# Autodesk Inventor assembly: leg_motor_moudle_MIR
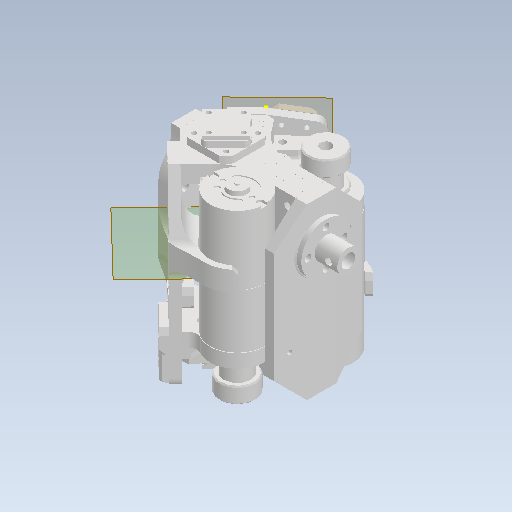
[picture p0: Inventor's stored thumbnail of the model, 512x512]
Saved by Autodesk Inventor 2020 (Build 240168000, 168)
## iProperties
Created: 2019-05-09
Part Number: leg_motor_moudle_MIR
Document SubType Name: Assembly
Designer: psrob
Author: psrob
## Documents named in this file (17)
- E:\projects-2\project dog gen2\hardware\leg_motor_moudle_MIR.iam
- E:\projects-2\project dog gen2\hardware\leg_basket_1_MIR.ipt
- E:\projects-2\project dog gen2\hardware\leg_basket_2_MIR.ipt
- E:\projects-2\project dog gen2\hardware\motor_holder_MIR.ipt
- E:\projects-2\project dog gen2\hardware\leg_basket_3_MIR.ipt
- E:\projects-2\project dog gen2\hardware\pin_3_14_MIR.ipt
- E:\projects-2\project dog gen2\hardware\motor_2_MIR.ipt
- E:\projects-2\project dog gen2\hardware\pin_6_20_MIR.ipt
- E:\projects-2\project dog gen2\hardware\pin_6_60_MIR.ipt
- E:\projects-2\project dog gen2\hardware\2GT_wheel_MIR.ipt
- E:\projects-2\project dog gen2\hardware\bearing_6_13_5_MIR.ipt
- E:\projects-2\project dog gen2\hardware\flange_6mm_MIR.ipt
- E:\projects-2\project dog gen2\hardware\cross_axis_holder_1_MIR.ipt
- E:\projects-2\project dog gen2\hardware\2GT_wheel_5_MIR.ipt
- E:\projects-2\project dog gen2\hardware\encoder_ass_MIR.iam
- E:\projects-2\project dog gen2\hardware\belt_holder_2_MIR.ipt
- E:\projects-2\project dog gen2\hardware\bearing_3_10_5.ipt
## Components (27 placed, 16 different names)
1. leg_basket_1_MIR:1 — Insert:6, Insert:5, Insert:8, Insert:7, Insert:2, Insert:1, Insert:4, Insert:3, Insert:29, Insert:28
2. leg_basket_2_MIR:1 — Insert:6, Insert:5, Insert:12, Insert:9, Insert:15, Insert:24, Insert:26, Insert:34, Insert:35
3. leg_basket_2_MIR:2 — Insert:8, Insert:7, Insert:11, Insert:10, Insert:14, Insert:25, Tangent:2, Mate:1, Insert:27, Insert:32, Insert:33
4. motor_holder_MIR:1 — Insert:2, Insert:1, Insert:20, Insert:19
5. motor_holder_MIR:2 — Insert:4, Insert:3, Insert:18, Insert:17
6. leg_basket_3_MIR:1 — Insert:12, Insert:11, Flush:1, Insert:36, Insert:37
7. leg_basket_3_MIR:2 — Insert:10, Insert:9, Insert:38, Insert:39
8. pin_3_14_MIR:2 — Insert:14
9. pin_3_14_MIR:4 — Insert:15
10. motor_2_MIR:1 — Insert:20, Insert:19, Insert:30
11. motor_2_MIR:2 — Insert:18, Insert:17, Insert:31
12. pin_6_20_MIR:1 — Insert:22
13. pin_6_60_MIR:1 — Insert:21, Insert:23, Tangent:1
14. 2GT_wheel_MIR:1 — Insert:21
15. bearing_6_13_5_MIR:1 — Insert:24, Insert:22
16. bearing_6_13_5_MIR:2 — Insert:25, Insert:23
17. flange_6mm_MIR:1 — Tangent:2, Tangent:1, Mate:1
18. cross_axis_holder_1_MIR:1 — Flush:1, Insert:27, Insert:26
19. flange_6mm_MIR:2 — Insert:29, Insert:28
20. 2GT_wheel_5_MIR:1 — Insert:31
21. 2GT_wheel_5_MIR:2 — Insert:30
22. encoder_ass_MIR:1 [sub-assembly] — Insert:32, Insert:33
23. encoder_ass_MIR:2 [sub-assembly] — Insert:34, Insert:35
24. belt_holder_2_MIR:1 — Insert:36, Insert:37, Insert:41
25. belt_holder_2_MIR:2 — Insert:38, Insert:39, Insert:40
26. bearing_3_10_5:1 — Insert:40
27. bearing_3_10_5:2 — Insert:41
## Relationships (43: Insert 39, Tangent 2, Mate 2)
- Insert:6: leg_basket_1_MIR:1 ↔ leg_basket_2_MIR:1
- Insert:5: leg_basket_1_MIR:1 ↔ leg_basket_2_MIR:1
- Insert:8: leg_basket_1_MIR:1 ↔ leg_basket_2_MIR:2
- Insert:7: leg_basket_1_MIR:1 ↔ leg_basket_2_MIR:2
- Insert:2: leg_basket_1_MIR:1 ↔ motor_holder_MIR:1
- Insert:1: leg_basket_1_MIR:1 ↔ motor_holder_MIR:1
- Insert:4: leg_basket_1_MIR:1 ↔ motor_holder_MIR:2
- Insert:3: leg_basket_1_MIR:1 ↔ motor_holder_MIR:2
- Insert:12: leg_basket_2_MIR:1 ↔ leg_basket_3_MIR:1
- Insert:11: leg_basket_2_MIR:2 ↔ leg_basket_3_MIR:1
- Insert:10: leg_basket_2_MIR:2 ↔ leg_basket_3_MIR:2
- Insert:9: leg_basket_2_MIR:1 ↔ leg_basket_3_MIR:2
- Insert:14: leg_basket_2_MIR:2 ↔ pin_3_14_MIR:2
- Insert:15: leg_basket_2_MIR:1 ↔ pin_3_14_MIR:4
- Insert:20: motor_holder_MIR:1 ↔ motor_2_MIR:1
- Insert:19: motor_holder_MIR:1 ↔ motor_2_MIR:1
- Insert:18: motor_holder_MIR:2 ↔ motor_2_MIR:2
- Insert:17: motor_holder_MIR:2 ↔ motor_2_MIR:2
- Insert:21 (-21 mm): pin_6_60_MIR:1 ↔ 2GT_wheel_MIR:1
- Insert:24: leg_basket_2_MIR:1 ↔ bearing_6_13_5_MIR:1
- Insert:22: pin_6_20_MIR:1 ↔ bearing_6_13_5_MIR:1
- Insert:25: leg_basket_2_MIR:2 ↔ bearing_6_13_5_MIR:2
- Insert:23: pin_6_60_MIR:1 ↔ bearing_6_13_5_MIR:2
- Tangent:2: leg_basket_2_MIR:2 ↔ flange_6mm_MIR:1
- Tangent:1: pin_6_60_MIR:1 ↔ flange_6mm_MIR:1
- Mate:1 (-5 mm): leg_basket_2_MIR:2 ↔ flange_6mm_MIR:1
- Flush:1 [Mate]: leg_basket_3_MIR:1 ↔ cross_axis_holder_1_MIR:1
- Insert:27: leg_basket_2_MIR:2 ↔ cross_axis_holder_1_MIR:1
- Insert:26: leg_basket_2_MIR:1 ↔ cross_axis_holder_1_MIR:1
- Insert:29: leg_basket_1_MIR:1 ↔ flange_6mm_MIR:2
- Insert:28: leg_basket_1_MIR:1 ↔ flange_6mm_MIR:2
- Insert:31 (-3 mm): motor_2_MIR:2 ↔ 2GT_wheel_5_MIR:1
- Insert:30 (-3 mm): motor_2_MIR:1 ↔ 2GT_wheel_5_MIR:2
- Insert:32: leg_basket_2_MIR:2 ↔ encoder_ass_MIR:1
- Insert:33: leg_basket_2_MIR:2 ↔ encoder_ass_MIR:1
- Insert:34: leg_basket_2_MIR:1 ↔ encoder_ass_MIR:2
- Insert:35: leg_basket_2_MIR:1 ↔ encoder_ass_MIR:2
- Insert:36: leg_basket_3_MIR:1 ↔ belt_holder_2_MIR:1
- Insert:37: leg_basket_3_MIR:1 ↔ belt_holder_2_MIR:1
- Insert:38: leg_basket_3_MIR:2 ↔ belt_holder_2_MIR:2
- Insert:39: leg_basket_3_MIR:2 ↔ belt_holder_2_MIR:2
- Insert:40: belt_holder_2_MIR:2 ↔ bearing_3_10_5:1
- Insert:41: belt_holder_2_MIR:1 ↔ bearing_3_10_5:2
